# Autodesk Inventor assembly: Assembly1
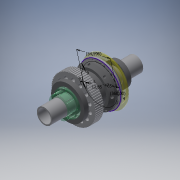
[picture p0: Inventor's stored thumbnail of the model, 180x180]
Saved by Autodesk Inventor 2018.1 (Build 221171000, 171)
## iProperties
Created: 2022-05-13
Part Number: Assembly1
Document SubType Name: Assembly
Designer: mouta
Author: mouta
## Documents named in this file (13)
- C:\Users\Bureau\Mon Drive\Manu\USINAGE\MoteurVelo\Arbre primaire\Assembly1.iam
- C:\Users\Bureau\Mon Drive\Manu\USINAGE\MoteurVelo\Arbre primaire\Axe manivelles.ipt
- C:\Users\Bureau\Mon Drive\Manu\USINAGE\MoteurVelo\Arbre primaire\bague pour roue libre.ipt
- C:\Users\Bureau\Mon Drive\Manu\USINAGE\MoteurVelo\Arbre primaire\roue libre.ipt
- C:\Users\Bureau\Mon Drive\Manu\USINAGE\MoteurVelo\Arbre primaire\roulement  25 32 4.ipt
- C:\Users\Bureau\Mon Drive\Manu\USINAGE\MoteurVelo\Arbre primaire\bague 25 32 16.ipt
- C:\Users\Bureau\Mon Drive\Manu\USINAGE\MoteurVelo\Arbre primaire\entraineur.ipt
- C:\Users\Bureau\Mon Drive\Manu\USINAGE\MoteurVelo\Arbre primaire\poulie 72 dents.ipt
- C:\Users\Bureau\Mon Drive\Manu\USINAGE\MoteurVelo\Arbre primaire\roulement 40 52 7.ipt
- C:\Users\Bureau\Mon Drive\Manu\USINAGE\MoteurVelo\Arbre primaire\roulement 25 37 7.ipt
- C:\Users\Bureau\Mon Drive\Manu\USINAGE\MoteurVelo\Arbre primaire\entraineur sur roue libre.ipt
- C:\Users\Bureau\Mon Drive\Manu\USINAGE\MoteurVelo\Arbre primaire\fin entraineur.ipt
- C:\Users\Bureau\Mon Drive\Manu\USINAGE\MoteurVelo\Arbre primaire\roue codeuse.ipt
## Components (12 placed, 12 different names)
1. Axe manivelles:1 — Mate:1, Flush:1, Mate:4, Flush:2, Mate:5, Mate:7, Mate:12, Mate:14, Flush:3, Mate:15, Mate:20, Mate:21
2. bague pour roue libre:1 — Mate:1, Flush:1, Mate:2, Mate:3
3. roue libre:1 — Mate:2, Mate:3, Mate:16, Mate:23
4. roulement  25 32 4:1 — Mate:4, Flush:2, Mate:6, Mate:8
5. bague 25 32 16:1 — Mate:5, Mate:6
6. entraineur:1 — Mate:7, Mate:8, Mate:13, Mate:22
7. poulie 72 dents:1 — Mate:21, Mate:22
8. roulement 40 52 7:1 — Mate:12, Mate:13
9. roulement 25 37 7:1 — Mate:14, Flush:3
10. entraineur sur roue libre:1 — Mate:15, Mate:16, Mate:17, Mate:18, Mate:19
11. fin entraineur:1 — Mate:17, Mate:18, Mate:19
12. roue codeuse:1 — Mate:20, Mate:23
## Relationships (23: Mate 20, Flush 3)
- Mate:1: Axe manivelles:1 ↔ bague pour roue libre:1
- Flush:1 (-42.9 mm): Axe manivelles:1 ↔ bague pour roue libre:1
- Mate:2: bague pour roue libre:1 ↔ roue libre:1
- Mate:3: bague pour roue libre:1 ↔ roue libre:1
- Mate:4: Axe manivelles:1 ↔ roulement  25 32 4:1
- Flush:2 (1 mm): Axe manivelles:1 ↔ roulement  25 32 4:1
- Mate:5: Axe manivelles:1 ↔ bague 25 32 16:1
- Mate:6: roulement  25 32 4:1 ↔ bague 25 32 16:1
- Mate:7: Axe manivelles:1 ↔ entraineur:1
- Mate:8: roulement  25 32 4:1 ↔ entraineur:1
- Mate:12: Axe manivelles:1 ↔ roulement 40 52 7:1
- Mate:13: entraineur:1 ↔ roulement 40 52 7:1
- Mate:14: Axe manivelles:1 ↔ roulement 25 37 7:1
- Flush:3 (-25 mm): Axe manivelles:1 ↔ roulement 25 37 7:1
- Mate:15: Axe manivelles:1 ↔ entraineur sur roue libre:1
- Mate:16: roue libre:1 ↔ entraineur sur roue libre:1
- Mate:17: entraineur sur roue libre:1 ↔ fin entraineur:1
- Mate:18: entraineur sur roue libre:1 ↔ fin entraineur:1
- Mate:19: entraineur sur roue libre:1 ↔ fin entraineur:1
- Mate:20: Axe manivelles:1 ↔ roue codeuse:1
- Mate:21: Axe manivelles:1 ↔ poulie 72 dents:1
- Mate:22: entraineur:1 ↔ poulie 72 dents:1
- Mate:23: roue libre:1 ↔ roue codeuse:1
